# Autodesk Inventor assembly: Anglerfish_bonne_mamman_m12large_v0
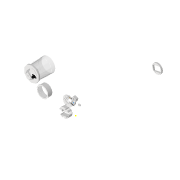
[picture p0: Inventor's stored thumbnail of the model, 180x180]
Saved by Autodesk Inventor 2022 (Build 260153000, 153)
## iProperties
Created: 2022-04-02
Part Number: Anglerfish_bonne_mamman_m12large_v0
Document SubType Name: Assembly
Designer: Prakash Lab
Author: Prakash Lab
## Documents named in this file (15)
- C:\Users\UC2\Documents\GitHub\Matchboxscope\INVENTOR\ANGLERFISH\Anglerfish_bonne_mamman_m12large_v0.iam
- C:\Users\UC2\Documents\GitHub\Matchboxscope\INVENTOR\ANGLERFISH\00_ESP3-CAM.iam
- C:\Users\UC2\Documents\GitHub\Matchboxscope\INVENTOR\ANGLERFISH\00_Powerbank.ipt
- C:\Users\diederichbenedict\Documents\Inventor\Content Center Files\R2022\de-DE\DIN 912\DIN 912 - M3 x 0.5 x 25 x 18.ipt
- C:\Users\UC2\Documents\GitHub\Matchboxscope\INVENTOR\ANGLERFISH\00_bonne_maman_jar.ipt
- C:\Users\UC2\Documents\GitHub\Matchboxscope\INVENTOR\ANGLERFISH\Anglerfish_Jar_Adapterplate_v1.ipt
- C:\Users\UC2\Documents\GitHub\Matchboxscope\INVENTOR\ANGLERFISH\Anglerfish_bottom_v0.ipt
- C:\Users\UC2\Documents\GitHub\Matchboxscope\INVENTOR\ANGLERFISH\Matchboxscope_M12_Lensadapter_v0.ipt
- C:\Users\UC2\Documents\GitHub\Matchboxscope\INVENTOR\ANGLERFISH\Anglerfish_Lightplate_Tosslink.ipt
- C:\Users\UC2\Documents\GitHub\Matchboxscope\INVENTOR\ANGLERFISH\00_toslink_launcher_v3.ipt
- C:\Users\UC2\Documents\GitHub\Matchboxscope\INVENTOR\ANGLERFISH\Anglerfish_Lightplate_Tislinkbridge.ipt
- C:\Users\UC2\Documents\GitHub\Matchboxscope\INVENTOR\ANGLERFISH\Anglerfish_middle2_m12VCMLens_large_v2.ipt
- C:\Users\UC2\Documents\GitHub\Matchboxscope\INVENTOR\ANGLERFISH\00_CCTV_M12_VCM_large.ipt
- C:\Users\UC2\Documents\GitHub\Matchboxscope\INVENTOR\ANGLERFISH\Anglerfish_spacer8mm_bottom_v0.ipt
- C:\Users\UC2\Documents\GitHub\Matchboxscope\INVENTOR\ANGLERFISH\Anglerfish_Lightplate_rotator.ipt
## Components (16 placed, 14 different names)
1. DIN 912 - ersetzt durch DIN EN ISO 4762 M3 x 25:5
2. DIN 912 - ersetzt durch DIN EN ISO 4762 M3 x 25:7
3. DIN 912 - ersetzt durch DIN EN ISO 4762 M3 x 25:8
4. 00_Powerbank:1
5. Anglerfish_Lightplate_Tislinkbridge:1 — Passend:14, Winkel:4, Passend:15
6. 00_toslink_launcher_v3:1
7. Anglerfish_Lightplate_Tosslink:1 — Passend:13, Winkel:3, Passend:14, Passend:15
8. Anglerfish_Lightplate_rotator:1 — Passend:11, Passend:12, Winkel:2, Passend:13, Winkel:4
9. 00_bonne_maman_jar:1 — Passend:10, Winkel:1, Fluchtend:1, Passend:11, Passend:12
10. Anglerfish_Jar_Adapterplate_v1:1
11. Anglerfish_bottom_v0:1
12. Anglerfish_spacer8mm_bottom_v0:1
13. Anglerfish_middle2_m12VCMLens_large_v2:1
14. 00_CCTV_M12_VCM_large:1
15. Matchboxscope_M12_Lensadapter_v0:1
16. 00_ESP3-CAM:1 [sub-assembly]
## Relationships (11: Mate 6, Angle 4, Flush 1)
- Passend:10 [Mate]: 00_bonne_maman_jar:1
- Winkel:1 [Angle] (0 deg): 00_bonne_maman_jar:1
- Fluchtend:1 [Flush]: 00_bonne_maman_jar:1
- Passend:11 [Mate]: Anglerfish_Lightplate_rotator:1 ↔ 00_bonne_maman_jar:1
- Passend:12 [Mate]: Anglerfish_Lightplate_rotator:1 ↔ 00_bonne_maman_jar:1
- Winkel:2 [Angle] (180 deg): Anglerfish_Lightplate_rotator:1
- Passend:13 [Mate]: Anglerfish_Lightplate_Tosslink:1 ↔ Anglerfish_Lightplate_rotator:1
- Winkel:3 [Angle] (0 deg): Anglerfish_Lightplate_Tosslink:1
- Passend:14 [Mate]: Anglerfish_Lightplate_Tislinkbridge:1 ↔ Anglerfish_Lightplate_Tosslink:1
- Winkel:4 [Angle] (155 deg): Anglerfish_Lightplate_Tislinkbridge:1 ↔ Anglerfish_Lightplate_rotator:1
- Passend:15 [Mate]: Anglerfish_Lightplate_Tislinkbridge:1 ↔ Anglerfish_Lightplate_Tosslink:1
